# Autodesk Inventor assembly: prototipo parte1
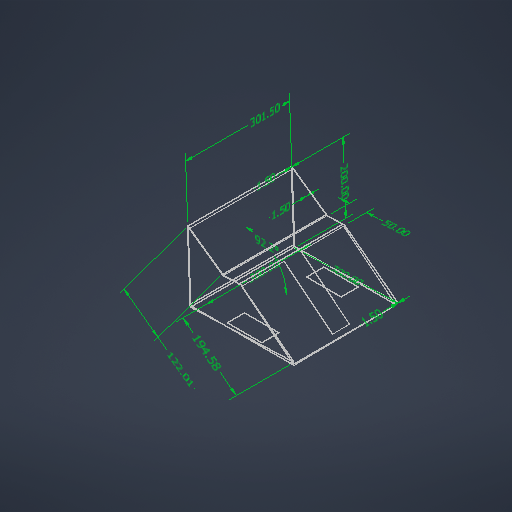
[picture p0: Inventor's stored thumbnail of the model, 512x512]
Saved by Autodesk Inventor 2027 (Build 310192060, 192F)
## iProperties
Created: 2026-09-04
Part Number: prototipo parte1
Document SubType Name: Assembly
Designer: Leandro
Author: Leandro
## Documents named in this file (7)
- C:\Users\Leandro\Desktop\battlebot\prototipo parte1.iam
- C:\Users\Leandro\Desktop\battlebot\base 30x30.ipt
- C:\Users\Leandro\Desktop\battlebot\parte lateral.ipt
- C:\Users\Leandro\Desktop\battlebot\parte trasera.ipt
- C:\Users\Leandro\Desktop\battlebot\panel frontal.ipt
- C:\Users\Leandro\Desktop\battlebot\recta.ipt
- C:\Users\Leandro\Desktop\battlebot\placa superior.ipt
## Components (7 placed, 6 different names)
1. base 30x30:1 — Coincidencia:1, Coincidencia:2
2. parte lateral:1 — Coincidencia:1, Coincidencia:4, Coincidencia:5
3. parte lateral:2 — Coincidencia:2, Coincidencia:3, Rígido:1
4. parte trasera:1 — Coincidencia:3
5. panel frontal:1
6. recta:1 — Coincidencia:4
7. placa superior:1 — Coincidencia:5, Rígido:1
## Relationships (6: Mate 5, WeldJoint 1)
- Coincidencia:1 [Mate]: base 30x30:1 ↔ parte lateral:1
- Coincidencia:2 [Mate]: base 30x30:1 ↔ parte lateral:2
- Coincidencia:3 [Mate]: parte lateral:2 ↔ parte trasera:1
- Coincidencia:4 [Mate]: parte lateral:1 ↔ recta:1
- Coincidencia:5 [Mate]: parte lateral:1 ↔ placa superior:1
- Rígido:1 [WeldJoint]: parte lateral:2 ↔ placa superior:1
